# Autodesk Inventor assembly: NEUROPIXELS GEN 1 PROBE ASSY
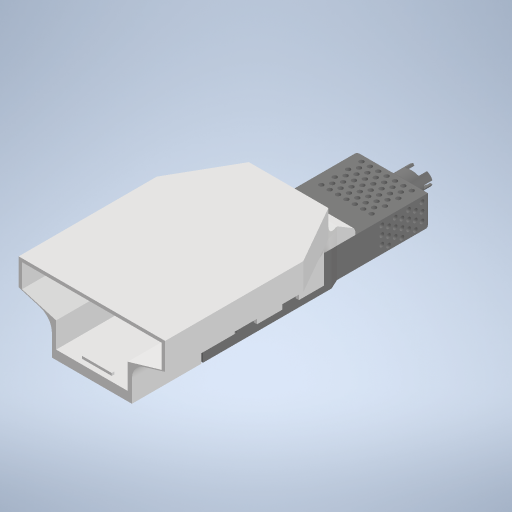
[picture p0: Inventor's stored thumbnail of the model, 512x512]
Saved by Autodesk Inventor 2023.4 (Build 274418000, 418)
## iProperties
RuleStatus: InUse
Created: 2019-08-15
Part Number: NEUROPIXELS GEN 1 PROBE ASSY
Document SubType Name: Assembly
Designer: mmelin
Sending System: Autodesk Inventor 2018
Preprocessor: ST-DEVELOPER v17
Title: C:\_WORKSPACE\DATA\PROJECTS\PROBE MOUNTS\MCAD\NEUROPIXELS GEN 1 PROBE ASSY.stp
Author: arnoldj
Revision Number: 0
## Documents named in this file (9)
- X:\chronic_holder\NP1\np1_full_assembly.iam
- X:\chronic_holder\imec_probe_files\np1_dovetail.ipt
- X:\chronic_holder\imec_probe_files\np1.ipt
- X:\chronic_holder\NP1\1_main_chassis\np1_main_chassis.ipt
- X:\chronic_holder\NP1\3_stereotax_holder\np1_stereotax_holder_part1.ipt
- X:\chronic_holder\NP1\3_stereotax_holder\np1_stereotax_holder_part2.ipt
- X:\chronic_holder\NP1\2_cap\cap_no_headstage\np1_cap_no_headstage.ipt
- X:\chronic_holder\NP1\2_cap\cap_with_headstage\np1_cap_with_headstage.ipt
- X:\chronic_holder\NP1\2_cap\cap_with_headstage\np1_headstage_cap_top_closure.ipt
## Components (8 placed, 8 different names)
1. NEUROPIXELS DOVE TAIL MOUNT:1 — Flush:1
2. NP2_FLEX_00-01:1
3. np1_main_chassis:1 — Flush:1, Flush:5, Flush:7, Flush:8, Flush:10, Flush:11, Flush:12, Flush:14, Flush:17, Flush:18, Flush:19, Flush:20, Flush:21, Flush:22
4. np1_stereotax_holder_part1:1 — Flush:5, Flush:7
5. np1_stereotax_holder_part2:1 — Flush:8, Flush:10
6. np1_cap_no_headstage:1 — Flush:11, Flush:18, Flush:19
7. np1_cap_with_headstage:1 — Flush:12, Flush:14, Flush:17, Flush:20, Flush:21, Flush:22, Flush:23, Flush:24
8. np1_headstage_cap_top_closure:1 — Flush:23, Flush:24
## Relationships (16: Flush 16)
- Flush:1: NEUROPIXELS DOVE TAIL MOUNT:1 ↔ np1_main_chassis:1
- Flush:5: np1_main_chassis:1 ↔ np1_stereotax_holder_part1:1
- Flush:7: np1_main_chassis:1 ↔ np1_stereotax_holder_part1:1
- Flush:8: np1_main_chassis:1 ↔ np1_stereotax_holder_part2:1
- Flush:10: np1_main_chassis:1 ↔ np1_stereotax_holder_part2:1
- Flush:11: np1_main_chassis:1 ↔ np1_cap_no_headstage:1
- Flush:12: np1_main_chassis:1 ↔ np1_cap_with_headstage:1
- Flush:14 (3.9878 mm): np1_main_chassis:1 ↔ np1_cap_with_headstage:1
- Flush:17: np1_main_chassis:1 ↔ np1_cap_with_headstage:1
- Flush:18: np1_main_chassis:1 ↔ np1_cap_no_headstage:1
- Flush:19: np1_main_chassis:1 ↔ np1_cap_no_headstage:1
- Flush:20: np1_main_chassis:1 ↔ np1_cap_with_headstage:1
- Flush:21: np1_main_chassis:1 ↔ np1_cap_with_headstage:1
- Flush:22: np1_main_chassis:1 ↔ np1_cap_with_headstage:1
- Flush:23: np1_cap_with_headstage:1 ↔ np1_headstage_cap_top_closure:1
- Flush:24: np1_cap_with_headstage:1 ↔ np1_headstage_cap_top_closure:1
